# Autodesk Inventor assembly: SansRotor
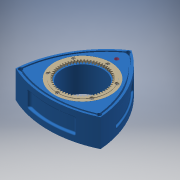
[picture p0: Inventor's stored thumbnail of the model, 180x180]
Saved by Autodesk Inventor 2019 (Build 230136000, 136)
## iProperties
Created: 2019-05-06
Part Number: SansRotor
Document SubType Name: Assembly
Designer: forev
Author: forev
## Documents named in this file (4)
- S:\Git_Repositories\Inventor_Projects\Wankel_Engine\SansRotor.iam
- S:\Univer\( G A C  ) Grafica asistată de calculator\Fișiere necesare\Fisiere necesare teme Inventor\6 - Wankel\Rotor.ipt
- S:\Univer\( G A C  ) Grafica asistată de calculator\Fișiere necesare\Fisiere necesare teme Inventor\6 - Wankel\Roata.ipt
- C:\Users\forev\Documents\Inventor\Content Center Files\R2019\en-US\ISO 4762(1)\DIN EN ISO 4762 - M3 x 5.ipt
## Components (8 placed, 3 different names)
1. Rotor:1 — Mate:1, Mate:2, Mate:3, Mate:4, Mate:5, Angle:1, Mate:6, Mate:7, Mate:8, Mate:9, Mate:10, Mate:11, Mate:12, Mate:13, Mate:14, Mate:15, Mate:16, Mate:17
2. Roata:1 — Mate:4, Mate:5, Angle:1
3. DIN EN ISO 4762 M3 x 5:1 — Mate:6, Mate:7
4. DIN EN ISO 4762 M3 x 5:2 — Mate:8, Mate:9
5. DIN EN ISO 4762 M3 x 5:3 — Mate:10, Mate:11
6. DIN EN ISO 4762 M3 x 5:4 — Mate:12, Mate:13
7. DIN EN ISO 4762 M3 x 5:5 — Mate:14, Mate:15
8. DIN EN ISO 4762 M3 x 5:6 — Mate:16, Mate:17
## Relationships (18: Mate 17, Angle 1)
- Mate:1: Rotor:1
- Mate:2: Rotor:1
- Mate:3: Rotor:1
- Mate:4: Rotor:1 ↔ Roata:1
- Mate:5: Rotor:1 ↔ Roata:1
- Angle:1 (0 deg): Rotor:1 ↔ Roata:1
- Mate:6: Rotor:1 ↔ DIN EN ISO 4762 M3 x 5:1
- Mate:7: Rotor:1 ↔ DIN EN ISO 4762 M3 x 5:1
- Mate:8: Rotor:1 ↔ DIN EN ISO 4762 M3 x 5:2
- Mate:9: Rotor:1 ↔ DIN EN ISO 4762 M3 x 5:2
- Mate:10: Rotor:1 ↔ DIN EN ISO 4762 M3 x 5:3
- Mate:11: Rotor:1 ↔ DIN EN ISO 4762 M3 x 5:3
- Mate:12: Rotor:1 ↔ DIN EN ISO 4762 M3 x 5:4
- Mate:13: Rotor:1 ↔ DIN EN ISO 4762 M3 x 5:4
- Mate:14: Rotor:1 ↔ DIN EN ISO 4762 M3 x 5:5
- Mate:15: Rotor:1 ↔ DIN EN ISO 4762 M3 x 5:5
- Mate:16: Rotor:1 ↔ DIN EN ISO 4762 M3 x 5:6
- Mate:17: Rotor:1 ↔ DIN EN ISO 4762 M3 x 5:6
